# Autodesk Inventor assembly: 50-J5
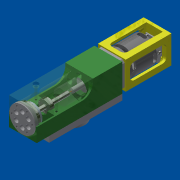
[picture p0: Inventor's stored thumbnail of the model, 180x180]
Saved by Autodesk Inventor 2018 (Build 220112000, 112)
## iProperties
Created: 2020-07-02
Part Number: 50-J5
Document SubType Name: Assembly
Designer: Bunny320
Author: Bunny320
## Documents named in this file (11)
- C:\Users\Bunny320\Desktop\sechs\4-CAD\50-J5.iam
- C:\Users\Bunny320\Desktop\sechs\4-CAD\motor unit 2820.iam
- C:\Users\Bunny320\Desktop\sechs\4-CAD\502-gearbox-housing.ipt
- C:\Users\Bunny320\Desktop\sechs\4-CAD\standardParts\W 606-2Z\W 606-2Z.iam
- C:\Users\Bunny320\Desktop\sechs\4-CAD\standardParts\61705-2RZ\W 61705-2RZ.iam
- C:\Users\Bunny320\Desktop\sechs\4-CAD\405-output disk.ipt
- C:\Users\Bunny320\Desktop\sechs\4-CAD\504-shaft.ipt
- C:\Users\Bunny320\Desktop\sechs\4-CAD\403-coupler dummy.ipt
- C:\Users\Bunny320\Desktop\sechs\4-CAD\standardParts\Pololu mounting hub\pololu-universal-aluminum-mounting-hub-for-6mm-shaft-m3-holes.ipt
- C:\Users\Bunny320\Desktop\sechs\4-CAD\501-flange.ipt
- C:\Users\Bunny320\Desktop\sechs\4-CAD\502-gearbox-housing-cap.ipt
## Components (10 placed, 10 different names)
1. motor unit 2820:1 [sub-assembly] — Flush:1, Flush:2, Flush:3, Mate:1, Mate:2, Mate:3, Mate:9, Mate:10
2. 502-gearbox-housing:1 — Mate:1, Mate:2, Mate:3, Mate:4, Mate:5, Mate:6, Flush:4, Mate:13, Mate:14, Mate:15, Mate:16, Mate:17, Mate:18
3. W 606-2Z:1 [sub-assembly] — Mate:4, Mate:5
4. W 61705-2RZ:1 [sub-assembly] — Mate:6, Mate:7, Mate:8, Flush:4
5. 405-output disk:1 — Mate:7, Mate:8, Mate:12
6. 504-shaft:1 — Mate:9, Mate:11
7. 403-coupler dummy:1 — Mate:10
8. pololu-universal-aluminum-mounting-hub-for-6mm-shaft-m3-holes:1 — Mate:11, Mate:12
9. 501-flange:1 — Mate:13, Mate:14, Mate:15
10. 502-gearbox-housing-cap:1 — Mate:16, Mate:17, Mate:18
## Relationships (22: Mate 18, Flush 4)
- Flush:1: motor unit 2820:1
- Flush:2: motor unit 2820:1
- Flush:3: motor unit 2820:1
- Mate:1: motor unit 2820:1 ↔ 502-gearbox-housing:1
- Mate:2: motor unit 2820:1 ↔ 502-gearbox-housing:1
- Mate:3: motor unit 2820:1 ↔ 502-gearbox-housing:1
- Mate:4: 502-gearbox-housing:1 ↔ W 606-2Z:1
- Mate:5: 502-gearbox-housing:1 ↔ W 606-2Z:1
- Mate:6: 502-gearbox-housing:1 ↔ W 61705-2RZ:1
- Mate:7: W 61705-2RZ:1 ↔ 405-output disk:1
- Mate:8: W 61705-2RZ:1 ↔ 405-output disk:1
- Flush:4: 502-gearbox-housing:1 ↔ W 61705-2RZ:1
- Mate:9: motor unit 2820:1 ↔ 504-shaft:1
- Mate:10: motor unit 2820:1 ↔ 403-coupler dummy:1
- Mate:11: 504-shaft:1 ↔ pololu-universal-aluminum-mounting-hub-for-6mm-shaft-m3-holes:1
- Mate:12: 405-output disk:1 ↔ pololu-universal-aluminum-mounting-hub-for-6mm-shaft-m3-holes:1
- Mate:13: 502-gearbox-housing:1 ↔ 501-flange:1
- Mate:14: 502-gearbox-housing:1 ↔ 501-flange:1
- Mate:15: 502-gearbox-housing:1 ↔ 501-flange:1
- Mate:16: 502-gearbox-housing:1 ↔ 502-gearbox-housing-cap:1
- Mate:17: 502-gearbox-housing:1 ↔ 502-gearbox-housing-cap:1
- Mate:18: 502-gearbox-housing:1 ↔ 502-gearbox-housing-cap:1
